# Autodesk Inventor assembly: Rear Panel
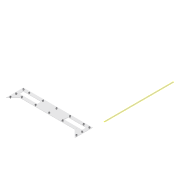
[picture p0: Inventor's stored thumbnail of the model, 180x180]
Saved by Autodesk Inventor 2017 (Build 210142000, 142)
## iProperties
Created: 2016-08-02
Part Number: Rear Panel
Document SubType Name: Assembly
Designer: User
Author: User
## Documents named in this file (3)
- C:\Autodesk\SL-Inventor\Rear Panel.iam
- C:\Autodesk\SL-Inventor\Acrylic-Back-Panel.ipt
- C:\Autodesk\SL-Inventor\BoltandTee.iam
## Components (16 placed, 2 different names)
1. Acrylic-Back-Panel:1
2. BoltandTee:1 [sub-assembly]
3. BoltandTee:2 [sub-assembly]
4. BoltandTee:3 [sub-assembly]
5. BoltandTee:4 [sub-assembly]
6. BoltandTee:5 [sub-assembly]
7. BoltandTee:6 [sub-assembly]
8. BoltandTee:7 [sub-assembly]
9. BoltandTee:8 [sub-assembly]
10. BoltandTee:9 [sub-assembly]
11. BoltandTee:10 [sub-assembly]
12. BoltandTee:11 [sub-assembly]
13. BoltandTee:12 [sub-assembly]
14. BoltandTee:13 [sub-assembly]
15. BoltandTee:14 [sub-assembly]
16. BoltandTee:15 [sub-assembly]
## Relationships (15: Insert 15)
- [Insert]: Acrylic-Back-Panel:1 ↔ BoltandTee:15
- [Insert]: Acrylic-Back-Panel:1 ↔ BoltandTee:14
- [Insert]: Acrylic-Back-Panel:1 ↔ BoltandTee:13
- [Insert]: Acrylic-Back-Panel:1 ↔ BoltandTee:12
- [Insert]: Acrylic-Back-Panel:1 ↔ BoltandTee:10
- [Insert]: Acrylic-Back-Panel:1 ↔ BoltandTee:11
- [Insert]: Acrylic-Back-Panel:1 ↔ BoltandTee:8
- [Insert]: Acrylic-Back-Panel:1 ↔ BoltandTee:9
- [Insert]: Acrylic-Back-Panel:1 ↔ BoltandTee:6
- [Insert]: Acrylic-Back-Panel:1 ↔ BoltandTee:7
- [Insert]: Acrylic-Back-Panel:1 ↔ BoltandTee:5
- [Insert]: Acrylic-Back-Panel:1 ↔ BoltandTee:4
- [Insert]: Acrylic-Back-Panel:1 ↔ BoltandTee:1
- [Insert]: Acrylic-Back-Panel:1 ↔ BoltandTee:2
- [Insert]: Acrylic-Back-Panel:1 ↔ BoltandTee:3
